# Autodesk Inventor assembly: Assembly1
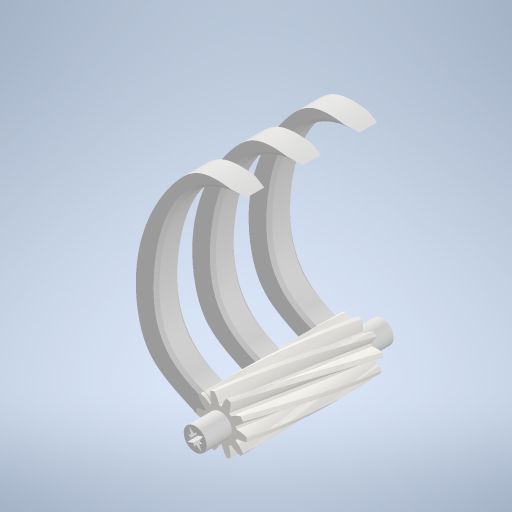
[picture p0: Inventor's stored thumbnail of the model, 512x512]
Saved by Autodesk Inventor 2024 (Build 280153000, 153)
## iProperties
Created: 2023-05-17
Part Number: Assembly1
Document SubType Name: Assembly
Designer: chris
Author: chris
## Documents named in this file (10)
- C:\Users\chris\Documents\biologically-inspired-perching-drone\hardware\Large_Scale_Claw\Version3\Assembly1.iam
- C:\Users\chris\Documents\biologically-inspired-perching-drone\hardware\Large_Scale_Claw\Version3\base.ipt
- C:\Users\chris\Documents\biologically-inspired-perching-drone\hardware\Large_Scale_Claw\Version3\3_arm.ipt
- C:\Users\chris\Documents\biologically-inspired-perching-drone\hardware\Large_Scale_Claw\Version3\2_arm.ipt
- C:\Users\chris\Documents\biologically-inspired-perching-drone\hardware\Large_Scale_Claw\Version3\Assembly1\Design Accelerator\Spur Gears1.iam
- C:\Users\chris\Documents\biologically-inspired-perching-drone\hardware\Large_Scale_Claw\Version3\wall_2.ipt
- C:\Users\chris\Documents\biologically-inspired-perching-drone\hardware\Large_Scale_Claw\Version3\shaft_collar.ipt
- C:\Users\chris\Downloads\pololu-universal-aluminum-mounting-hub-for-3mm-shaft-m3-holes\pololu-universal-aluminum-mounting-hub-for-3mm-shaft-m3-holes.ipt
- C:\Users\chris\Downloads\micro-metal-gearmotor-backshaft\micro-metal-gearmotor-backshaft.ipt
- C:\Users\chris\Downloads\20d-metal-gearmotors-3d-models\20d-metal-gearmotor-25-31\20d-metal-gearmotor-25-31.ipt
## Components (10 placed, 9 different names)
1. base:1 — Flush:8, Flush:11, Flush:15, Flush:16, Flush:17, Flush:18
2. 3_arm:1 — Mate:8, Mate:11, Mate:23
3. 2_arm:1 — Flush:12, Mate:13, Mate:14, Mate:24
4. Spur Gears:1 [sub-assembly] — Mate:23, Mate:24, Mate:25, Mate:26
5. wall_2:1 — Flush:8, Flush:9, Symmetry:1, Mate:11, Mate:19, Flush:18, Mate:25, Mate:26
6. wall_2:2 — Flush:9, Flush:11, Symmetry:1, Flush:15, Flush:16, Flush:17
7. shaft_collar:1 — Mate:13, Mate:14, Mate:15, Mate:20, Mate:21, Mate:22
8. pololu-universal-aluminum-mounting-hub-for-3mm-shaft-m3-holes:1 — Mate:15, Mate:18, Mate:20
9. micro-metal-gearmotor-backshaft:1 — Mate:18, Mate:19, Mate:21
10. 20d-metal-gearmotor-25-31:1 — Mate:22
## Relationships (23: Mate 14, Flush 8, Symmetry 1)
- Flush:8: base:1 ↔ wall_2:1
- Flush:9: wall_2:1 ↔ wall_2:2
- Flush:11: base:1 ↔ wall_2:2
- Symmetry:1: wall_2:1 ↔ wall_2:2
- Mate:8: 3_arm:1
- Flush:12: 2_arm:1
- Mate:11: 3_arm:1 ↔ wall_2:1
- Mate:13: 2_arm:1 ↔ shaft_collar:1
- Mate:14: 2_arm:1 ↔ shaft_collar:1
- Mate:15: shaft_collar:1 ↔ pololu-universal-aluminum-mounting-hub-for-3mm-shaft-m3-holes:1
- Mate:18: pololu-universal-aluminum-mounting-hub-for-3mm-shaft-m3-holes:1 ↔ micro-metal-gearmotor-backshaft:1
- Mate:19: wall_2:1 ↔ micro-metal-gearmotor-backshaft:1
- Mate:20: shaft_collar:1 ↔ pololu-universal-aluminum-mounting-hub-for-3mm-shaft-m3-holes:1
- Mate:21: shaft_collar:1 ↔ micro-metal-gearmotor-backshaft:1
- Mate:22: shaft_collar:1 ↔ 20d-metal-gearmotor-25-31:1
- Flush:15: base:1 ↔ wall_2:2
- Flush:16: base:1 ↔ wall_2:2
- Flush:17: base:1 ↔ wall_2:2
- Flush:18: base:1 ↔ wall_2:1
- Mate:23: 3_arm:1 ↔ Spur Gears:1
- Mate:24: 2_arm:1 ↔ Spur Gears:1
- Mate:25 (0.5 mm): Spur Gears:1 ↔ wall_2:1
- Mate:26 (0.5 mm): Spur Gears:1 ↔ wall_2:1
